# Autodesk Inventor assembly: Electrronic Enclosure
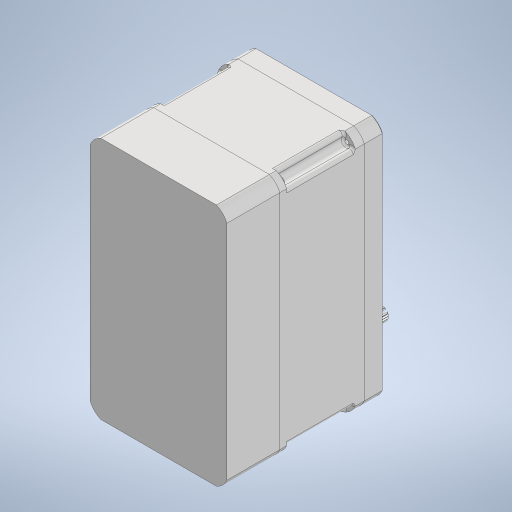
[picture p0: Inventor's stored thumbnail of the model, 512x512]
Saved by Autodesk Inventor 2023 (Build 270158000, 158)
## iProperties
Created: 2021-02-17
Part Number: Electrronic Enclosure
Document SubType Name: Assembly
Designer: jeffb
Sending System: Autodesk Translation Framework v9.7.0.1280
Preprocessor: ST-DEVELOPER v18.1
Title: /Users/emac5k/Dropbox/Adafruit/3D/Adafruit_CAD_Parts/4741 OLED 1.5in/Adafruit Grayscale 1.5-inch 128x128 OLED v2.step
## Documents named in this file (11)
- F:\OneDrive\Documents\Inventor\ELS\Electrronic Enclosure.iam
- F:\OneDrive\Documents\Inventor\ELS\1.5 inch oled\PCB Component.iam
- F:\OneDrive\Documents\Inventor\ELS\Encoder\4991 QT Rotary Encoder.iam
- F:\OneDrive\Documents\Inventor\ELS\878 7-segment display backpack.ipt
- F:\OneDrive\Documents\Inventor\ELS\main board\ELS Main Board.iam
- F:\OneDrive\Documents\Inventor\ELS\Housing Bottom.ipt
- F:\OneDrive\Documents\Inventor\ELS\96817A300_Thread-Forming Screws for Thin Plastic.ipt
- F:\OneDrive\Documents\Inventor\ELS\Housing Top.ipt
- F:\OneDrive\Documents\Inventor\ELS\96001A124_Torx Plus Rounded Head Thread-Forming Screws.ipt
- F:\OneDrive\Documents\Inventor\ELS\Oled Mount.ipt
- F:\OneDrive\Documents\Inventor\ELS\Housing Middle.ipt
## Components (37 placed, 10 different names)
1. PCB Component:1 [sub-assembly] — Angle:1, Angle:4, Flush:1, Angle:5, Angle:6, Mate:2, Mate:3, Mate:4, Mate:5, Flush:10, Flush:11, Flush:12, Flush:13
2. 4991 QT Rotary Encoder:1 [sub-assembly] — Angle:1, Angle:4, Mate:4, Flush:7, Mate:6, Angle:7, Insert:11, Insert:12, Insert:13, Insert:14
3. 878 7-segment display backpack:1 — Flush:1, Mate:1, Mate:2, Mate:3, Flush:3, Insert:6, Insert:7, Insert:8, Insert:9
4. ELS Main Board:1 [sub-assembly] — Angle:5, Angle:6, Mate:1, Flush:3, Flush:7, Mate:5, Flush:8, Flush:9, Insert:1, Insert:3, Insert:4, Insert:5
5. Housing Bottom:1 — Flush:8, Flush:9, Flush:14, Flush:15
6. 96817A300_Thread-Forming Screws for Thin Plastic:2 — Insert:1
7. 96817A300_Thread-Forming Screws for Thin Plastic:3 — Insert:4
8. 96817A300_Thread-Forming Screws for Thin Plastic:4 — Insert:3
9. 96817A300_Thread-Forming Screws for Thin Plastic:5 — Insert:5
10. Housing Top:1 — Flush:10, Flush:11, Mate:6, Insert:10, Insert:19, Insert:20, Insert:21, Insert:22, Insert:27, Insert:28, Insert:29, Insert:30
11. 96001A124_Torx Plus Rounded Head Thread-Forming Screws:1 — Insert:6
12. 96001A124_Torx Plus Rounded Head Thread-Forming Screws:2 — Insert:7
13. 96001A124_Torx Plus Rounded Head Thread-Forming Screws:3 — Insert:9
14. 96001A124_Torx Plus Rounded Head Thread-Forming Screws:4 — Insert:8
15. 4991 QT Rotary Encoder:2 [sub-assembly] — Angle:7, Insert:10, Insert:15, Insert:16, Insert:17, Insert:18
16. 96001A124_Torx Plus Rounded Head Thread-Forming Screws:5 — Insert:18
17. 96001A124_Torx Plus Rounded Head Thread-Forming Screws:6 — Insert:17
18. 96001A124_Torx Plus Rounded Head Thread-Forming Screws:7 — Insert:12
19. 96001A124_Torx Plus Rounded Head Thread-Forming Screws:8 — Insert:11
20. 96001A124_Torx Plus Rounded Head Thread-Forming Screws:9 — Insert:16
21. 96001A124_Torx Plus Rounded Head Thread-Forming Screws:10 — Insert:15
22. 96001A124_Torx Plus Rounded Head Thread-Forming Screws:11 — Insert:14
23. 96001A124_Torx Plus Rounded Head Thread-Forming Screws:12 — Insert:13
24. Oled Mount:1 — Flush:12, Flush:13
25. 96001A124_Torx Plus Rounded Head Thread-Forming Screws:13 — Insert:19
26. 96001A124_Torx Plus Rounded Head Thread-Forming Screws:14 — Insert:20
27. 96001A124_Torx Plus Rounded Head Thread-Forming Screws:15 — Insert:21
28. 96001A124_Torx Plus Rounded Head Thread-Forming Screws:16 — Insert:22
29. Housing Middle:1 — Flush:14, Flush:15, Insert:23, Insert:24, Insert:25, Insert:26
30. 96001A124_Torx Plus Rounded Head Thread-Forming Screws:17 — Insert:24
31. 96001A124_Torx Plus Rounded Head Thread-Forming Screws:18 — Insert:23
32. 96001A124_Torx Plus Rounded Head Thread-Forming Screws:19 — Insert:25
33. 96001A124_Torx Plus Rounded Head Thread-Forming Screws:20 — Insert:26
34. 96001A124_Torx Plus Rounded Head Thread-Forming Screws:21 — Insert:28
35. 96001A124_Torx Plus Rounded Head Thread-Forming Screws:22 — Insert:27
36. 96001A124_Torx Plus Rounded Head Thread-Forming Screws:23 — Insert:30
37. 96001A124_Torx Plus Rounded Head Thread-Forming Screws:24 — Insert:29
## Relationships (51: Insert 29, Flush 11, Mate 6, Angle 5)
- Angle:1 (0 deg): PCB Component:1 ↔ 4991 QT Rotary Encoder:1
- Angle:4 (0 deg): PCB Component:1 ↔ 4991 QT Rotary Encoder:1
- Flush:1: PCB Component:1 ↔ 878 7-segment display backpack:1
- Angle:5 (0 deg): PCB Component:1 ↔ ELS Main Board:1
- Angle:6 (0 deg): PCB Component:1 ↔ ELS Main Board:1
- Mate:1 (38.1 mm): 878 7-segment display backpack:1 ↔ ELS Main Board:1
- Mate:2 (3 mm): PCB Component:1 ↔ 878 7-segment display backpack:1
- Mate:3: PCB Component:1 ↔ 878 7-segment display backpack:1
- Mate:4 (1 mm): PCB Component:1 ↔ 4991 QT Rotary Encoder:1
- Flush:3: 878 7-segment display backpack:1 ↔ ELS Main Board:1
- Flush:7: 4991 QT Rotary Encoder:1 ↔ ELS Main Board:1
- Mate:5: PCB Component:1 ↔ ELS Main Board:1
- Flush:8: ELS Main Board:1 ↔ Housing Bottom:1
- Flush:9: ELS Main Board:1 ↔ Housing Bottom:1
- Insert:1: ELS Main Board:1 ↔ 96817A300_Thread-Forming Screws for Thin Plastic:2
- Insert:3: ELS Main Board:1 ↔ 96817A300_Thread-Forming Screws for Thin Plastic:4
- Insert:4: ELS Main Board:1 ↔ 96817A300_Thread-Forming Screws for Thin Plastic:3
- Insert:5: ELS Main Board:1 ↔ 96817A300_Thread-Forming Screws for Thin Plastic:5
- Flush:10: PCB Component:1 ↔ Housing Top:1
- Flush:11: PCB Component:1 ↔ Housing Top:1
- Mate:6: 4991 QT Rotary Encoder:1 ↔ Housing Top:1
- Insert:6: 878 7-segment display backpack:1 ↔ 96001A124_Torx Plus Rounded Head Thread-Forming Screws:1
- Insert:7: 878 7-segment display backpack:1 ↔ 96001A124_Torx Plus Rounded Head Thread-Forming Screws:2
- Insert:8: 878 7-segment display backpack:1 ↔ 96001A124_Torx Plus Rounded Head Thread-Forming Screws:4
- Insert:9: 878 7-segment display backpack:1 ↔ 96001A124_Torx Plus Rounded Head Thread-Forming Screws:3
- Angle:7 (0 deg): 4991 QT Rotary Encoder:1 ↔ 4991 QT Rotary Encoder:2
- Insert:10: Housing Top:1 ↔ 4991 QT Rotary Encoder:2
- Insert:11: 4991 QT Rotary Encoder:1 ↔ 96001A124_Torx Plus Rounded Head Thread-Forming Screws:8
- Insert:12: 4991 QT Rotary Encoder:1 ↔ 96001A124_Torx Plus Rounded Head Thread-Forming Screws:7
- Insert:13: 4991 QT Rotary Encoder:1 ↔ 96001A124_Torx Plus Rounded Head Thread-Forming Screws:12
- Insert:14: 4991 QT Rotary Encoder:1 ↔ 96001A124_Torx Plus Rounded Head Thread-Forming Screws:11
- Insert:15: 4991 QT Rotary Encoder:2 ↔ 96001A124_Torx Plus Rounded Head Thread-Forming Screws:10
- Insert:16: 4991 QT Rotary Encoder:2 ↔ 96001A124_Torx Plus Rounded Head Thread-Forming Screws:9
- Insert:17: 4991 QT Rotary Encoder:2 ↔ 96001A124_Torx Plus Rounded Head Thread-Forming Screws:6
- Insert:18: 4991 QT Rotary Encoder:2 ↔ 96001A124_Torx Plus Rounded Head Thread-Forming Screws:5
- Flush:12: PCB Component:1 ↔ Oled Mount:1
- Flush:13: PCB Component:1 ↔ Oled Mount:1
- Insert:19: Housing Top:1 ↔ 96001A124_Torx Plus Rounded Head Thread-Forming Screws:13
- Insert:20: Housing Top:1 ↔ 96001A124_Torx Plus Rounded Head Thread-Forming Screws:14
- Insert:21: Housing Top:1 ↔ 96001A124_Torx Plus Rounded Head Thread-Forming Screws:15
- Insert:22: Housing Top:1 ↔ 96001A124_Torx Plus Rounded Head Thread-Forming Screws:16
- Flush:14: Housing Bottom:1 ↔ Housing Middle:1
- Flush:15: Housing Bottom:1 ↔ Housing Middle:1
- Insert:23: Housing Middle:1 ↔ 96001A124_Torx Plus Rounded Head Thread-Forming Screws:18
- Insert:24: Housing Middle:1 ↔ 96001A124_Torx Plus Rounded Head Thread-Forming Screws:17
- Insert:25: Housing Middle:1 ↔ 96001A124_Torx Plus Rounded Head Thread-Forming Screws:19
- Insert:26: Housing Middle:1 ↔ 96001A124_Torx Plus Rounded Head Thread-Forming Screws:20
- Insert:27: Housing Top:1 ↔ 96001A124_Torx Plus Rounded Head Thread-Forming Screws:22
- Insert:28: Housing Top:1 ↔ 96001A124_Torx Plus Rounded Head Thread-Forming Screws:21
- Insert:29: Housing Top:1 ↔ 96001A124_Torx Plus Rounded Head Thread-Forming Screws:24
- Insert:30: Housing Top:1 ↔ 96001A124_Torx Plus Rounded Head Thread-Forming Screws:23
